# Autodesk Inventor assembly: FullFrame.002
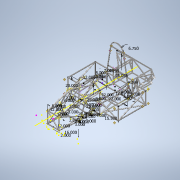
[picture p0: Inventor's stored thumbnail of the model, 180x180]
Saved by Autodesk Inventor 2021 (Build 250183000, 183)
## iProperties
_SolveAssemblyDoc: Frame Generator Solve Assembly
_Version: 25.0.0
Created: 2020-11-09
Part Number: FullFrame.002
Document SubType Name: Assembly
Designer: qv17m
Author: qv17m
## Documents named in this file (4)
- C:\Users\qv17m\Documents\Inventor\FSAE\FullCarV1.5.3\FullCarV1.5.3\FullFrame.002\FullFrame.002.iam
- C:\Users\qv17m\Documents\Inventor\FSAE\FullCarV1.5.3\FullCarV1.5.3\FullFrame.002\FrameMembers\Frame 1604946896143.iam
- C:\Users\qv17m\Documents\Inventor\FSAE\FullCarV1.5.3\FullCarV1.5.3\FullFrame.002\RearFrame.002.ipt
- C:\Users\qv17m\Documents\Inventor\FSAE\FullCarV1.5.3\FullCarV1.5.3\FullFrame.002\FrontFrame.002.ipt
## Components (3 placed, 3 different names)
1. RearFrame.002:1 — Mate:1
2. FrontFrame.002:1 — Mate:1
3. Frame 1604946896143:1 [sub-assembly]
## Relationships (1: Mate 1)
- Mate:1: RearFrame.002:1 ↔ FrontFrame.002:1
